# Autodesk Inventor assembly: Assembly4
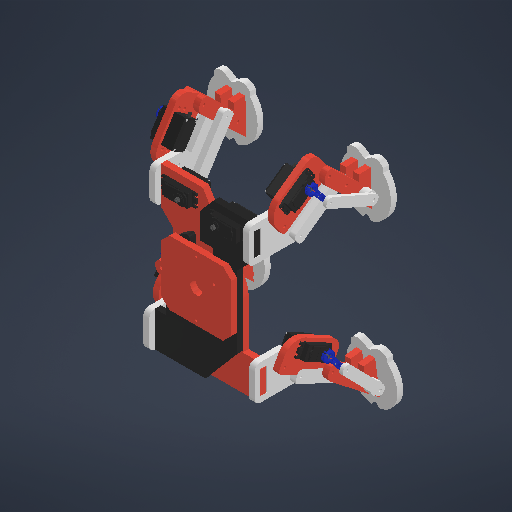
[picture p0: Inventor's stored thumbnail of the model, 512x512]
Saved by Autodesk Inventor 2026.2 (Build 302298010, 298A)
## iProperties
Created: 2026-05-09
Part Number: Assembly4
Document SubType Name: Assembly
Designer: Martina
Author: Martina
## Documents named in this file (32)
- D:\Semester 4\Praktikum Robotika\Project Robotika\Project Robotika\Assembly4.iam
- D:\Semester 4\Praktikum Robotika\Project Robotika\Project Robotika\Body Slider Merah\slider merah.ipt
- D:\Semester 4\Praktikum Robotika\Project Robotika\Project Robotika\Body Slider Hitam\Component4.ipt
- D:\Semester 4\Praktikum Robotika\Project Robotika\Project Robotika\Body Kaki Servo\Component2.ipt
- D:\Semester 4\Praktikum Robotika\Project Robotika\Project Robotika\Body Lengan Kaki\Component2.ipt
- D:\Semester 4\Praktikum Robotika\Project Robotika\Project Robotika\Atas Slider.ipt
- D:\Semester 4\Praktikum Robotika\Project Robotika\YouCanBuildDog-main\YouCanBuildDog-main\CAD\dog02_large\dog02_large\Buat Ulang\Hip.ipt
- D:\Semester 4\Praktikum Robotika\Project Robotika\YouCanBuildDog-main\YouCanBuildDog-main\CAD\dog02_large\dog02_large\Buat Ulang\LegLver.ipt
- D:\Semester 4\Praktikum Robotika\Project Robotika\YouCanBuildDog-main\YouCanBuildDog-main\CAD\dog02_large\dog02_large\Buat Ulang\Spacer6.ipt
- D:\Semester 4\Praktikum Robotika\Project Robotika\YouCanBuildDog-main\YouCanBuildDog-main\CAD\dog02_large\dog02_large\Buat Ulang\Uleg01.ipt
- D:\Semester 4\Praktikum Robotika\Project Robotika\Project Robotika\telapak kaki.ipt
- D:\Semester 4\Praktikum Robotika\Project Robotika\Project Robotika\Body Kaki Servo\Component2_MIR.ipt
- D:\Semester 4\Praktikum Robotika\Project Robotika\Project Robotika\Body Lengan Kaki\Component2_MIR.ipt
- D:\Semester 4\Praktikum Robotika\Project Robotika\YouCanBuildDog-main\YouCanBuildDog-main\CAD\dog02_large\dog02_large\Buat Ulang\Spacer6_MIR.ipt
- D:\Semester 4\Praktikum Robotika\Project Robotika\YouCanBuildDog-main\YouCanBuildDog-main\CAD\dog02_large\dog02_large\Buat Ulang\Uleg01_MIR.ipt
- D:\Semester 4\Praktikum Robotika\Project Robotika\YouCanBuildDog-main\YouCanBuildDog-main\CAD\dog02_large\dog02_large\Buat Ulang\LegLver_MIR.ipt
- D:\Semester 4\Praktikum Robotika\Project Robotika\Project Robotika\telapak kaki_MIR.ipt
- D:\Semester 4\Praktikum Robotika\Project Robotika\Project Robotika\Body Kaki Servo\Component2_MIR1.ipt
- D:\Semester 4\Praktikum Robotika\Project Robotika\Project Robotika\Body Lengan Kaki\Component2_MIR1.ipt
- D:\Semester 4\Praktikum Robotika\Project Robotika\YouCanBuildDog-main\YouCanBuildDog-main\CAD\dog02_large\dog02_large\Buat Ulang\Spacer6_MIR1.ipt
- D:\Semester 4\Praktikum Robotika\Project Robotika\YouCanBuildDog-main\YouCanBuildDog-main\CAD\dog02_large\dog02_large\Buat Ulang\Uleg01_MIR1.ipt
- D:\Semester 4\Praktikum Robotika\Project Robotika\YouCanBuildDog-main\YouCanBuildDog-main\CAD\dog02_large\dog02_large\Buat Ulang\LegLver_MIR1.ipt
- D:\Semester 4\Praktikum Robotika\Project Robotika\Project Robotika\telapak kaki_MIR1.ipt
- D:\Semester 4\Praktikum Robotika\Project Robotika\Project Robotika\Body Kaki Servo\Component2_MIR_MIR.ipt
- D:\Semester 4\Praktikum Robotika\Project Robotika\Project Robotika\Body Lengan Kaki\Component2_MIR_MIR.ipt
- D:\Semester 4\Praktikum Robotika\Project Robotika\YouCanBuildDog-main\YouCanBuildDog-main\CAD\dog02_large\dog02_large\Buat Ulang\Spacer6_MIR_MIR.ipt
- D:\Semester 4\Praktikum Robotika\Project Robotika\YouCanBuildDog-main\YouCanBuildDog-main\CAD\dog02_large\dog02_large\Buat Ulang\Uleg01_MIR_MIR.ipt
- D:\Semester 4\Praktikum Robotika\Project Robotika\YouCanBuildDog-main\YouCanBuildDog-main\CAD\dog02_large\dog02_large\Buat Ulang\LegLver_MIR_MIR.ipt
- D:\Semester 4\Praktikum Robotika\Project Robotika\Project Robotika\telapak kaki_MIR_MIR.ipt
- D:\Semester 4\Praktikum Robotika\Project Robotika\Project Robotika\hip hitam.ipt
- C:\Users\Martina\Downloads\MG995\MG995.iam
- D:\Semester 4\Praktikum Robotika\Project Robotika\YouCanBuildDog-main\YouCanBuildDog-main\CAD\dog02_large\smart dustbin part 3 (aliminum clam) v3.ipt
## Components (49 placed, 27 different names)
1. slider merah:1 — Mate:25, Mate:26, Mate:27, Mate:28, Mate:29, Mate:30, Mate:69, Mate:70, Mate:71, Mate:97, Mate:98, Mate:99, Mate:100
2. Component4:1 — Mate:60, Mate:61, Mate:62, Mate:63, Mate:64, Mate:65, Mate:66, Mate:67, Mate:68, Mate:69, Mate:70, Mate:71, Mate:93, Mate:94, Mate:95, Mate:96
3. Atas Slider:1 — Mate:66, Mate:67, Mate:68
4. Hip:1 — Mate:28, Mate:29, Mate:30, Rotational:21, Rotational:22, Mate:31
5. Component2:10 — Rotational:20, Rotational:21, Mate:76, Mate:77, Mate:78, Mate:79
6. Component2:11
7. Spacer6:4
8. Uleg01:4 — Mate:80
9. LegLver:7 — Mate:31
10. telapak kaki:4
11. Component2:12 — Rotational:20
12. LegLver:8 — Rotational:22
13. Hip:2 — Mate:25, Mate:26, Mate:27, Rotational:28, Mate:38, Mate:39
14. Component2_MIR:1 — Rotational:26, Rotational:28, Mate:85, Mate:86, Mate:87, Mate:88
15. Component2_MIR:2 — Mate:32, Mate:33, Mate:34, Rotational:23, Rotational:25
16. Spacer6_MIR:1 — Rotational:23, Rotational:24
17. Uleg01_MIR:1 — Rotational:24, Mate:102
18. LegLver_MIR:1 — Rotational:25, Mate:38
19. telapak kaki_MIR:1 — Mate:32, Mate:33, Mate:34, Mate:35, Mate:36, Mate:37
20. Component2_MIR:3 — Mate:35, Mate:36, Mate:37, Rotational:26, Rotational:27
21. LegLver_MIR:2 — Rotational:27, Mate:39
22. Component2_MIR1:1 — Rotational:33, Rotational:43, Mate:89, Mate:90, Mate:91, Mate:92
23. Component2_MIR1:2 — Mate:44, Mate:45, Mate:46, Rotational:30, Rotational:32
24. Spacer6_MIR1:1 — Rotational:30, Rotational:31
25. Uleg01_MIR1:1 — Rotational:31, Mate:103
26. LegLver_MIR1:1 — Rotational:32, Mate:73
27. telapak kaki_MIR1:1 — Mate:44, Mate:45, Mate:46, Mate:47, Mate:48, Mate:49
28. Component2_MIR1:3 — Mate:47, Mate:48, Mate:49, Rotational:33, Rotational:35
29. LegLver_MIR1:2 — Rotational:35, Mate:72
30. Component2_MIR_MIR:1 — Rotational:40, Rotational:42, Mate:81, Mate:82, Mate:83, Mate:84
31. Component2_MIR_MIR:2 — Mate:54, Mate:55, Mate:56, Rotational:37, Rotational:39
32. Spacer6_MIR_MIR:1 — Rotational:37, Rotational:38
33. Uleg01_MIR_MIR:1 — Rotational:38, Mate:101
34. LegLver_MIR_MIR:1 — Rotational:39, Mate:75
35. telapak kaki_MIR_MIR:1 — Mate:54, Mate:55, Mate:56, Mate:57, Mate:58, Mate:59
36. Component2_MIR_MIR:3 — Mate:57, Mate:58, Mate:59, Rotational:40, Rotational:41
37. LegLver_MIR_MIR:2 — Rotational:41, Mate:74
38. hip hitam:1 — Mate:60, Mate:61, Mate:62, Rotational:43, Mate:72, Mate:73
39. hip hitam:2 — Mate:63, Mate:64, Mate:65, Rotational:42, Mate:74, Mate:75
40. MG995:1 [sub-assembly] — Mate:76, Mate:77, Mate:78, Mate:79, Insert:1
41. MG995:2 [sub-assembly] — Mate:81, Mate:82, Mate:83, Mate:84, Insert:2
42. MG995:3 [sub-assembly] — Mate:93, Mate:94, Mate:95, Mate:96
43. MG995:4 [sub-assembly] — Mate:97, Mate:98, Mate:99, Mate:100
44. MG995:5 [sub-assembly] — Mate:85, Mate:86, Mate:87, Mate:88, Insert:3
45. MG995:6 [sub-assembly] — Mate:89, Mate:90, Mate:91, Mate:92, Insert:4
46. smart dustbin part 3 (aliminum clam) v3:1 — Insert:1, Mate:80
47. smart dustbin part 3 (aliminum clam) v3:2 — Insert:4, Mate:103
48. smart dustbin part 3 (aliminum clam) v3:3 — Insert:3, Mate:102
49. smart dustbin part 3 (aliminum clam) v3:5 — Insert:2, Mate:101
## Relationships (106: Mate 77, RevoluteJoint 25, Insert 4)
- [RevoluteJoint]: Component2:11 ↔ Spacer6:4
- [RevoluteJoint]: Spacer6:4 ↔ Uleg01:4
- [Mate]: Component2:11 ↔ telapak kaki:4
- [Mate]: Component2:11 ↔ telapak kaki:4
- [Mate]: Component2:11 ↔ telapak kaki:4
- [Mate]: telapak kaki:4 ↔ Component2:12
- [Mate]: telapak kaki:4 ↔ Component2:12
- [Mate]: telapak kaki:4 ↔ Component2:12
- [RevoluteJoint] (-1 mm): Component2:11 ↔ LegLver:7
- [RevoluteJoint] (-1 mm): Component2:12 ↔ LegLver:8
- Mate:25: slider merah:1 ↔ Hip:2
- Mate:26: slider merah:1 ↔ Hip:2
- Mate:27: slider merah:1 ↔ Hip:2
- Mate:28: slider merah:1 ↔ Hip:1
- Mate:29: slider merah:1 ↔ Hip:1
- Mate:30: slider merah:1 ↔ Hip:1
- Rotational:20 [RevoluteJoint] (1 mm): Component2:10 ↔ Component2:12
- Rotational:21 [RevoluteJoint] (-1 mm): Hip:1 ↔ Component2:10
- Rotational:22 [RevoluteJoint] (1 mm): Hip:1 ↔ LegLver:8
- Mate:31 (-1.1 mm): Hip:1 ↔ LegLver:7
- Mate:32: Component2_MIR:2 ↔ telapak kaki_MIR:1
- Mate:33: Component2_MIR:2 ↔ telapak kaki_MIR:1
- Mate:34: Component2_MIR:2 ↔ telapak kaki_MIR:1
- Mate:35: telapak kaki_MIR:1 ↔ Component2_MIR:3
- Mate:36: telapak kaki_MIR:1 ↔ Component2_MIR:3
- Mate:37: telapak kaki_MIR:1 ↔ Component2_MIR:3
- Rotational:23 [RevoluteJoint]: Component2_MIR:2 ↔ Spacer6_MIR:1
- Rotational:24 [RevoluteJoint]: Spacer6_MIR:1 ↔ Uleg01_MIR:1
- Rotational:25 [RevoluteJoint] (1 mm): Component2_MIR:2 ↔ LegLver_MIR:1
- Rotational:26 [RevoluteJoint] (-1 mm): Component2_MIR:1 ↔ Component2_MIR:3
- Rotational:27 [RevoluteJoint] (1 mm): Component2_MIR:3 ↔ LegLver_MIR:2
- Rotational:28 [RevoluteJoint] (1 mm): Hip:2 ↔ Component2_MIR:1
- Mate:38 (1.1 mm): Hip:2 ↔ LegLver_MIR:1
- Mate:39 (-1 mm): Hip:2 ↔ LegLver_MIR:2
- Mate:44: Component2_MIR1:2 ↔ telapak kaki_MIR1:1
- Mate:45: Component2_MIR1:2 ↔ telapak kaki_MIR1:1
- Mate:46: Component2_MIR1:2 ↔ telapak kaki_MIR1:1
- Mate:47: telapak kaki_MIR1:1 ↔ Component2_MIR1:3
- Mate:48: telapak kaki_MIR1:1 ↔ Component2_MIR1:3
- Mate:49: telapak kaki_MIR1:1 ↔ Component2_MIR1:3
- Mate:54: Component2_MIR_MIR:2 ↔ telapak kaki_MIR_MIR:1
- Mate:55: Component2_MIR_MIR:2 ↔ telapak kaki_MIR_MIR:1
- Mate:56: Component2_MIR_MIR:2 ↔ telapak kaki_MIR_MIR:1
- Mate:57: telapak kaki_MIR_MIR:1 ↔ Component2_MIR_MIR:3
- Mate:58: telapak kaki_MIR_MIR:1 ↔ Component2_MIR_MIR:3
- Mate:59: telapak kaki_MIR_MIR:1 ↔ Component2_MIR_MIR:3
- Rotational:30 [RevoluteJoint]: Component2_MIR1:2 ↔ Spacer6_MIR1:1
- Rotational:31 [RevoluteJoint]: Spacer6_MIR1:1 ↔ Uleg01_MIR1:1
- Rotational:32 [RevoluteJoint] (1 mm): Component2_MIR1:2 ↔ LegLver_MIR1:1
- Rotational:33 [RevoluteJoint] (-1 mm): Component2_MIR1:1 ↔ Component2_MIR1:3
- Rotational:35 [RevoluteJoint] (1 mm): Component2_MIR1:3 ↔ LegLver_MIR1:2
- Rotational:37 [RevoluteJoint]: Component2_MIR_MIR:2 ↔ Spacer6_MIR_MIR:1
- Rotational:38 [RevoluteJoint]: Spacer6_MIR_MIR:1 ↔ Uleg01_MIR_MIR:1
- Rotational:39 [RevoluteJoint] (-1 mm): Component2_MIR_MIR:2 ↔ LegLver_MIR_MIR:1
- Rotational:40 [RevoluteJoint] (1 mm): Component2_MIR_MIR:1 ↔ Component2_MIR_MIR:3
- Rotational:41 [RevoluteJoint] (-1 mm): Component2_MIR_MIR:3 ↔ LegLver_MIR_MIR:2
- Mate:60: Component4:1 ↔ hip hitam:1
- Mate:61: Component4:1 ↔ hip hitam:1
- Mate:62: Component4:1 ↔ hip hitam:1
- Mate:63: Component4:1 ↔ hip hitam:2
- Mate:64: Component4:1 ↔ hip hitam:2
- Mate:65: Component4:1 ↔ hip hitam:2
- Mate:66 (-0.882 mm): Component4:1 ↔ Atas Slider:1
- Mate:67 (0.882 mm): Component4:1 ↔ Atas Slider:1
- Mate:68 (31.502 mm): Component4:1 ↔ Atas Slider:1
- Mate:69: slider merah:1 ↔ Component4:1
- Mate:70: slider merah:1 ↔ Component4:1
- Mate:71: slider merah:1 ↔ Component4:1
- Rotational:42 [RevoluteJoint] (-1 mm): Component2_MIR_MIR:1 ↔ hip hitam:2
- Rotational:43 [RevoluteJoint] (1 mm): Component2_MIR1:1 ↔ hip hitam:1
- Mate:72 (-1 mm): LegLver_MIR1:2 ↔ hip hitam:1
- Mate:73 (1.1 mm): LegLver_MIR1:1 ↔ hip hitam:1
- Mate:74 (1 mm): LegLver_MIR_MIR:2 ↔ hip hitam:2
- Mate:75 (1.1 mm): LegLver_MIR_MIR:1 ↔ hip hitam:2
- Mate:76: Component2:10 ↔ MG995:1
- Mate:77: Component2:10 ↔ MG995:1
- Mate:78: Component2:10 ↔ MG995:1
- Mate:79: Component2:10 ↔ MG995:1
- Insert:1 (0.1 mm): MG995:1 ↔ smart dustbin part 3 (aliminum clam) v3:1
- Mate:80: Uleg01:4 ↔ smart dustbin part 3 (aliminum clam) v3:1
- Mate:81: Component2_MIR_MIR:1 ↔ MG995:2
- Mate:82: Component2_MIR_MIR:1 ↔ MG995:2
- Mate:83: Component2_MIR_MIR:1 ↔ MG995:2
- Mate:84: Component2_MIR_MIR:1 ↔ MG995:2
- Insert:2 (0.1 mm): MG995:2 ↔ smart dustbin part 3 (aliminum clam) v3:5
- Mate:85: Component2_MIR:1 ↔ MG995:5
- Mate:86: Component2_MIR:1 ↔ MG995:5
- Mate:87: Component2_MIR:1 ↔ MG995:5
- Mate:88: Component2_MIR:1 ↔ MG995:5
- Mate:89: Component2_MIR1:1 ↔ MG995:6
- Mate:90: Component2_MIR1:1 ↔ MG995:6
- Mate:91: Component2_MIR1:1 ↔ MG995:6
- Mate:92: Component2_MIR1:1 ↔ MG995:6
- Mate:93: Component4:1 ↔ MG995:3
- Mate:94: Component4:1 ↔ MG995:3
- Mate:95: Component4:1 ↔ MG995:3
- Mate:96: Component4:1 ↔ MG995:3
- Mate:97: slider merah:1 ↔ MG995:4
- Mate:98: slider merah:1 ↔ MG995:4
- Mate:99: slider merah:1 ↔ MG995:4
- Mate:100: slider merah:1 ↔ MG995:4
- Insert:3 (-0.1 mm): MG995:5 ↔ smart dustbin part 3 (aliminum clam) v3:3
- Mate:101: Uleg01_MIR_MIR:1 ↔ smart dustbin part 3 (aliminum clam) v3:5
- Mate:102: Uleg01_MIR:1 ↔ smart dustbin part 3 (aliminum clam) v3:3
- Insert:4 (-0.1 mm): MG995:6 ↔ smart dustbin part 3 (aliminum clam) v3:2
- Mate:103: Uleg01_MIR1:1 ↔ smart dustbin part 3 (aliminum clam) v3:2
## Named parameters: d51_d0 = 0 mm, d52_d1 = 62.315981 deg, d53_d2 = 0 mm, d54_d3 = 19.914518 deg, d55_d4 = 0 mm, d56_d5 = 0 mm, d57_d6 = 0 mm, d58_d7 = 0 mm, d59_d8 = 0 mm, d60_d9 = 0 mm, d61_d13 = -1 mm, d62_d14 = -76.515723 deg, d63_d15 = -1 mm, d64_d16 = -166.515722 deg
